# Autodesk Inventor assembly: A1-18002-400-00 1.25in bar tube cap
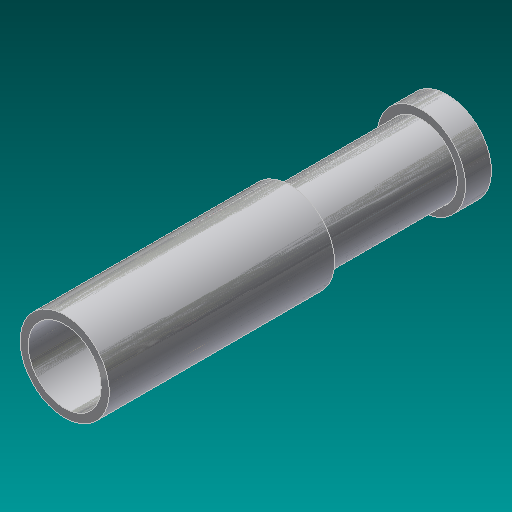
[picture p0: Inventor's stored thumbnail of the model, 512x512]
Saved by Autodesk Inventor 2017 (Build 210142000, 142)
## iProperties
Created: 2018-01-23
Part Number: A1-18002-400-00 1.25in bar tube cap
Document SubType Name: Assembly
Designer: Graeme_Van_Dongen
Mass: 386.057 g
Surface Area: 1079.24 cm^2
Volume: 275.755 cm^3
Density: 1.4 g/cm^3
Author: Graeme_Van_Dongen
## Documents named in this file (5)
- N:\A1 - Projects\A1-18\A1-18002--Alco Line boring skid\A1-18002-400-00 1.25in bar tube cap.iam
- N:\A1 - Projects\A1-18\A1-18002--Alco Line boring skid\A1-18002-100-34 1.25in bar tube end.ipt
- N:\A1 - Projects\A1-18\A1-18002--Alco Line boring skid\A1-18002-100-35 1.25in bar tube socket.ipt
- N:\A1 - Projects\A1-18\A1-18002--Alco Line boring skid\A1-18002-100-36 1.5in pipe cap.ipt
- A1-18002-100-36 1.5in pipe cap.ipt
## Components (3 placed, 3 different names)
1. A1-18002-100-34 1.25in bar tube end:1 — Insert:1, Angle:1, Insert:2, Angle:2
2. A1-18002-100-35 1.25in bar tube socket:1 — Insert:1, Angle:1
3. A1-18002-100-36 1.5in pipe cap:1 — Insert:2, Angle:2
## Relationships (4: Insert 2, Angle 2)
- Insert:1 (-50.8 mm): A1-18002-100-34 1.25in bar tube end:1 ↔ A1-18002-100-35 1.25in bar tube socket:1
- Angle:1 (0 deg): A1-18002-100-34 1.25in bar tube end:1 ↔ A1-18002-100-35 1.25in bar tube socket:1
- Insert:2: A1-18002-100-34 1.25in bar tube end:1 ↔ A1-18002-100-36 1.5in pipe cap:1
- Angle:2 (0 deg): A1-18002-100-34 1.25in bar tube end:1 ↔ A1-18002-100-36 1.5in pipe cap:1
